# Autodesk Inventor assembly: Assembly1
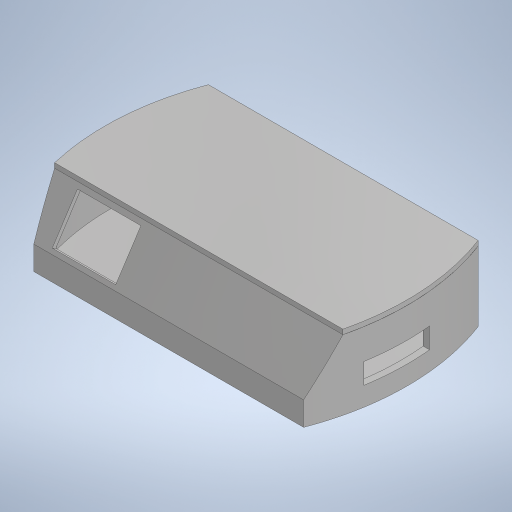
[picture p0: Inventor's stored thumbnail of the model, 512x512]
Saved by Autodesk Inventor 2023 (Build 270158000, 158)
## iProperties
Created: 2022-12-17
Part Number: Assembly1
Document SubType Name: Assembly
Designer: Aakif
Author: Aakif
## Documents named in this file (3)
- D:\Materi\Sem 5\Assembly1.iam
- D:\Materi\Sem 5\Earthquake Detector_Case v1.ipt
- D:\Materi\Sem 5\tutup.ipt
## Components (2 placed, 2 different names)
1. Earthquake Detector_Case v1:1 — Mate:1, Flush:1, Mate:2
2. tutup:1 — Mate:1, Flush:1, Mate:2
## Relationships (3: Mate 2, Flush 1)
- Mate:1: Earthquake Detector_Case v1:1 ↔ tutup:1
- Flush:1: Earthquake Detector_Case v1:1 ↔ tutup:1
- Mate:2: Earthquake Detector_Case v1:1 ↔ tutup:1
